# Autodesk Inventor assembly: arms
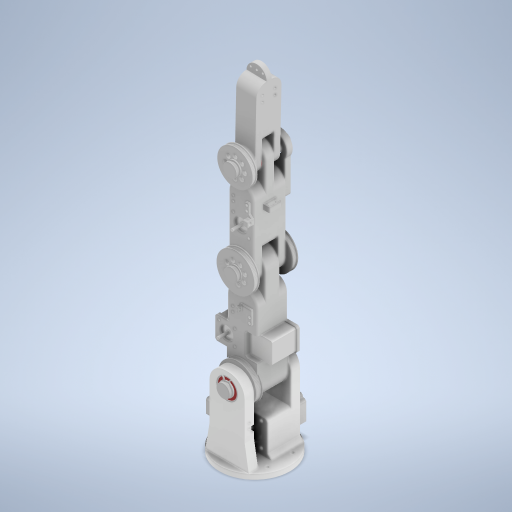
[picture p0: Inventor's stored thumbnail of the model, 512x512]
Saved by Autodesk Inventor 2024 (Build 280153000, 153)
## iProperties
Created: 2024-02-21
Part Number: arms
Document SubType Name: Assembly
Designer: MaartenGeorgesBuelen
Mass: 3190 g
Surface Area: 4481.69 cm^2
Volume: 2343.49 cm^3
Density: 1.36122 g/cm^3
Author: MaartenGeorgesBuelen
## Documents named in this file (26)
- C:\Users\MaartenGeorgesBuelen\Documents\Inventor\robot arm\arms\arms.iam
- C:\Users\MaartenGeorgesBuelen\Documents\Inventor\robot arm\base-new\base.ipt
- C:\Users\MaartenGeorgesBuelen\Documents\Inventor\robot arm\arms\lower arm with pulley.iam
- C:\Users\MaartenGeorgesBuelen\Documents\Inventor\robot arm\motors\stepper motor large.ipt
- C:\Users\MaartenGeorgesBuelen\Documents\Inventor\robot arm\hardware\pulley-small.ipt
- C:\Users\MaartenGeorgesBuelen\Documents\Inventor\robot arm\hardware\arm-bearings.ipt
- C:\Users\MaartenGeorgesBuelen\Documents\Inventor\robot arm\arms\arm middle.ipt
- C:\Users\MaartenGeorgesBuelen\Documents\Inventor\robot arm\arms\middle arm pulley.ipt
- C:\Users\MaartenGeorgesBuelen\Documents\Inventor\robot arm\motors\stepper motor.ipt
- C:\Users\MaartenGeorgesBuelen\Documents\Inventor\robot arm\upper arm.ipt
- C:\Users\MaartenGeorgesBuelen\Documents\Inventor\robot arm\arms\upper arm pulley.ipt
- C:\Users\MaartenGeorgesBuelen\Documents\Inventor\robot arm\arms\axle.ipt
- C:\Users\MaartenGeorgesBuelen\Documents\Inventor\robot arm\arms\base-tensioner.ipt
- C:\Users\MaartenGeorgesBuelen\Documents\Inventor\robot arm\arms\base-tensioner-head.ipt
- C:\Users\MaartenGeorgesBuelen\Documents\Inventor\robot arm\stl\bearing-holder.ipt
- C:\Users\MaartenGeorgesBuelen\Documents\Inventor\robot arm\hardware\axle_cap.ipt
- C:\Users\MaartenGeorgesBuelen\Documents\Inventor\robot arm\arms\bearing-spacer-middle.ipt
- C:\Users\MaartenGeorgesBuelen\Documents\Inventor\robot arm\arms\bearing-spacer-top.ipt
- C:\Users\MaartenGeorgesBuelen\Documents\Inventor\robot arm\arms\midle-tensioner.ipt
- C:\Users\MaartenGeorgesBuelen\Documents\Inventor\robot arm\arms\midle-tensioner_MIR.ipt
- C:\Users\MaartenGeorgesBuelen\Documents\Inventor\robot arm\arms\axle-middle.ipt
- C:\Users\MaartenGeorgesBuelen\Documents\Inventor\robot arm\arms\axle-upper.ipt
- C:\Users\MaartenGeorgesBuelen\Documents\Inventor\robot arm\arms\top-tensioner.ipt
- C:\Users\MaartenGeorgesBuelen\Documents\Inventor\robot arm\case\cable-clip.ipt
- C:\Users\MaartenGeorgesBuelen\Documents\Inventor\robot arm\arms\bearing for tensioner head.ipt
- C:\Users\MaartenGeorgesBuelen\Documents\Inventor\robot arm\stl\3rd arm support.ipt
## Components (33 placed, 25 different names)
1. base:1 — Rotational:1, Mate:9, Mate:10, Mate:11, Mate:14, Mate:28, Mate:29, Mate:30, Mate:31, Flush:7, Flush:8, Symmetry:1, Flush:10, Flush:35, Mate:35
2. lower arm with pulley:1 [sub-assembly] — Rotational:1, Mate:13, Flush:2, Flush:3, Flush:4, Mate:20, Mate:21, Mate:22, Mate:23, Flush:37, Flush:39
3. arm middle:1 — Flush:2, Mate:17, Flush:5, Mate:24, Mate:25, Mate:26, Flush:6, Flush:38, Flush:41, Flush:42, Flush:43
4. middle arm pulley:1
5. middle arm pulley:2 — Mate:17, Flush:40
6. stepper motor:3 — Flush:5, Mate:24
7. arm-bearings:5 — Mate:25
8. arm-bearings:6 — Mate:26
9. upper arm:1 — Flush:6, Mate:27, Mate:34
10. upper arm pulley:1 — Mate:27
11. axle:1 — Flush:7, Flush:36
12. base-tensioner:1 — Flush:8, Symmetry:1, Flush:10, Flush:34, Flush:44
13. base-tensioner-head:1 — Flush:34, Mate:32, Mate:33, Flush:44, Mate:35
14. bearing-holder:1 — Flush:35
15. axle_cap:1 — Flush:36
16. bearing-spacer-middle:1 — Flush:37
17. bearing-spacer-top:1 — Flush:38
18. midle-tensioner:1 — Flush:39
19. midle-tensioner_MIR:1
20. axle-middle:1 — Flush:40
21. axle-upper:1 — Mate:34
22. top-tensioner:1 — Flush:41
23. cable-clip:1 — Flush:42
24. bearing for tensioner head:1 — Mate:32, Mate:33
25. 3rd arm support:1 — Flush:43
26. stepper motor large:1 — Mate:8, Flush:1, Mate:9, Mate:10, Mate:11, Mate:29, Mate:30, Mate:31
27. pulley-small:1 — Mate:8, Flush:1
28. stepper motor:1 — Flush:4, Mate:21, Mate:23
29. stepper motor:2 — Flush:3, Mate:20, Mate:22
30. arm-bearings:1
31. arm-bearings:2 — Mate:13
32. arm-bearings:3 — Mate:14
33. arm-bearings:4 — Mate:28
## Relationships (45: Mate 23, Flush 20, RevoluteJoint 1, Symmetry 1)
- Rotational:1 [RevoluteJoint]: base:1 ↔ lower arm with pulley:1
- Mate:8: stepper motor large:1 ↔ pulley-small:1
- Flush:1: stepper motor large:1 ↔ pulley-small:1
- Mate:9: base:1 ↔ stepper motor large:1
- Mate:10: base:1 ↔ stepper motor large:1
- Mate:11: base:1 ↔ stepper motor large:1
- Mate:13: lower arm with pulley:1 ↔ arm-bearings:2
- Mate:14: base:1 ↔ arm-bearings:3
- Flush:2: lower arm with pulley:1 ↔ arm middle:1
- Mate:17: arm middle:1 ↔ middle arm pulley:2
- Flush:3 (6 mm): lower arm with pulley:1 ↔ stepper motor:2
- Flush:4 (6 mm): lower arm with pulley:1 ↔ stepper motor:1
- Mate:20 (-21 mm): lower arm with pulley:1 ↔ stepper motor:2
- Mate:21 (-21 mm): lower arm with pulley:1 ↔ stepper motor:1
- Mate:22 (2 mm): lower arm with pulley:1 ↔ stepper motor:2
- Mate:23 (2 mm): lower arm with pulley:1 ↔ stepper motor:1
- Flush:5 (6 mm): arm middle:1 ↔ stepper motor:3
- Mate:24 (-46 mm): arm middle:1 ↔ stepper motor:3
- Mate:25: arm middle:1 ↔ arm-bearings:5
- Mate:26: arm middle:1 ↔ arm-bearings:6
- Flush:6: arm middle:1 ↔ upper arm:1
- Mate:27: upper arm:1 ↔ upper arm pulley:1
- Mate:28: base:1 ↔ arm-bearings:4
- Mate:29 (2.5 mm): base:1 ↔ stepper motor large:1
- Mate:30 (2.5 mm): base:1 ↔ stepper motor large:1
- Mate:31: base:1 ↔ stepper motor large:1
- Flush:7: base:1 ↔ axle:1
- Flush:8: base:1 ↔ base-tensioner:1
- Symmetry:1: base:1 ↔ base-tensioner:1
- Flush:10: base:1 ↔ base-tensioner:1
- Flush:34: base-tensioner:1 ↔ base-tensioner-head:1
- Flush:35: base:1 ↔ bearing-holder:1
- Flush:36: axle:1 ↔ axle_cap:1
- Flush:37: lower arm with pulley:1 ↔ bearing-spacer-middle:1
- Flush:38: arm middle:1 ↔ bearing-spacer-top:1
- Flush:39: lower arm with pulley:1 ↔ midle-tensioner:1
- Flush:40: middle arm pulley:2 ↔ axle-middle:1
- Flush:41: arm middle:1 ↔ top-tensioner:1
- Flush:42: arm middle:1 ↔ cable-clip:1
- Mate:32: base-tensioner-head:1 ↔ bearing for tensioner head:1
- Mate:33: base-tensioner-head:1 ↔ bearing for tensioner head:1
- Mate:34: upper arm:1 ↔ axle-upper:1
- Flush:43: arm middle:1 ↔ 3rd arm support:1
- Flush:44 (1 mm): base-tensioner:1 ↔ base-tensioner-head:1
- Mate:35 (10.5 mm): base:1 ↔ base-tensioner-head:1
